# Autodesk Inventor assembly: Dropdown_Assembly_V3_Complete
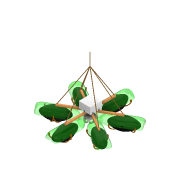
[picture p0: Inventor's stored thumbnail of the model, 180x180]
Saved by Autodesk Inventor 2021 (Build 250183000, 183)
## iProperties
Created: 2020-07-21
Part Number: Dropdown_Assembly_V3_Complete
Document SubType Name: Assembly
Designer: cameron
Mass: 991.522 g
Surface Area: 13651.5 cm^2
Volume: 1179.19 cm^3
Density: 0.840851 g/cm^3
Author: cameron
## Documents named in this file (10)
- C:\Users\camer\Git\Sure2020-DropdownSystem\InventorDropsonde\Dropdown_Assembly_V3_Complete.iam
- C:\Users\camer\Git\Sure2020-DropdownSystem\InventorDropsonde\PVC center piece.ipt
- C:\Users\camer\Git\Sure2020-DropdownSystem\InventorDropsonde\Dropdown_Assembly_V3.iam
- C:\Users\camer\Git\Sure2020-DropdownSystem\InventorDropsonde\Top rods.ipt
- C:\Users\camer\Git\Sure2020-DropdownSystem\InventorDropsonde\PCB housing.ipt
- C:\Users\camer\Git\Sure2020-DropdownSystem\InventorDropsonde\C brace.ipt
- C:\Users\camer\Git\Sure2020-DropdownSystem\InventorDropsonde\Balloon_Rope.ipt
- C:\Users\camer\OneDrive\Documents\Inventor\Content Center Files\R2021\en-US\AS 1427(04)\AS 1427 - M2.5 x 5(5) I.ipt
- C:\Users\camer\Git\Sure2020-DropdownSystem\InventorDropsonde\Staples.ipt
- C:\Users\camer\Git\Sure2020-DropdownSystem\InventorDropsonde\PCB_model_V5.ipt
## Components (29 placed, 9 different names)
1. PVC center piece:1 — Mate:1, Mate:2
2. Top rods:1 — Tangent:1, Tangent:2, Mate:3, Mate:4, Mate:6, Mate:8, Mate:10, Mate:12, Mate:14, Flush:1, Flush:2, Flush:10
3. PCB housing:1 — Mate:3, Mate:5, Mate:7, Mate:9, Mate:11, Mate:13, Mate:15, Mate:22
4. C brace:1 — Mate:10, Mate:11, Mate:16, Flush:7
5. C brace:2 — Mate:12, Mate:13, Mate:17, Flush:6
6. C brace:3 — Mate:4, Mate:5, Mate:18, Flush:8
7. C brace:4 — Mate:6, Mate:7, Mate:19, Flush:9
8. C brace:5 — Mate:8, Mate:9, Mate:20, Flush:4
9. C brace:6 — Mate:14, Mate:15, Mate:21, Flush:5
10. Balloon_Rope:1 — Flush:2, Flush:3
11. AS 1427 H - Metric M2.5 x 5:1 — Mate:16, Flush:7
12. AS 1427 H - Metric M2.5 x 5:2 — Mate:17, Flush:6
13. AS 1427 H - Metric M2.5 x 5:3 — Mate:18, Flush:8
14. AS 1427 H - Metric M2.5 x 5:4 — Mate:19, Flush:9
15. AS 1427 H - Metric M2.5 x 5:5 — Mate:20, Flush:4
16. AS 1427 H - Metric M2.5 x 5:6 — Mate:21, Flush:5
17. PCB_model_V5:1 — Mate:22
18. Dropdown_Assembly_V3:1 [sub-assembly] — Mate:1, Mate:2
19. Dropdown_Assembly_V3:2 [sub-assembly] — Tangent:2
20. Dropdown_Assembly_V3:3 [sub-assembly]
21. Dropdown_Assembly_V3:4 [sub-assembly] — Tangent:1
22. Dropdown_Assembly_V3:5 [sub-assembly]
23. Dropdown_Assembly_V3:6 [sub-assembly]
24. Staples:1 — Flush:11, Flush:12
25. Staples:2
26. Staples:3
27. Staples:4
28. Staples:5
29. Staples:6
## Component patterns: (6 elements, first: Dropdown_Assembly_V3:1), (6 elements, first: Staples:1)
## Relationships (36: Mate 22, Flush 12, Tangent 2)
- Mate:1: PVC center piece:1 ↔ Dropdown_Assembly_V3:1
- Mate:2: PVC center piece:1 ↔ Dropdown_Assembly_V3:1
- Tangent:1: Top rods:1 ↔ Dropdown_Assembly_V3:4
- Tangent:2: Top rods:1 ↔ Dropdown_Assembly_V3:2
- Mate:3 (1 mm): Top rods:1 ↔ PCB housing:1
- Mate:4: Top rods:1 ↔ C brace:3
- Mate:5: PCB housing:1 ↔ C brace:3
- Mate:6: Top rods:1 ↔ C brace:4
- Mate:7: PCB housing:1 ↔ C brace:4
- Mate:8: Top rods:1 ↔ C brace:5
- Mate:9: PCB housing:1 ↔ C brace:5
- Mate:10: Top rods:1 ↔ C brace:1
- Mate:11: PCB housing:1 ↔ C brace:1
- Mate:12: Top rods:1 ↔ C brace:2
- Mate:13: PCB housing:1 ↔ C brace:2
- Mate:14: Top rods:1 ↔ C brace:6
- Mate:15: PCB housing:1 ↔ C brace:6
- Flush:1 (300 mm): Top rods:1
- Flush:2: Top rods:1 ↔ Balloon_Rope:1
- Flush:3: Balloon_Rope:1
- Mate:16: C brace:1 ↔ AS 1427 H - Metric M2.5 x 5:1
- Mate:17: C brace:2 ↔ AS 1427 H - Metric M2.5 x 5:2
- Mate:18: C brace:3 ↔ AS 1427 H - Metric M2.5 x 5:3
- Mate:19: C brace:4 ↔ AS 1427 H - Metric M2.5 x 5:4
- Mate:20: C brace:5 ↔ AS 1427 H - Metric M2.5 x 5:5
- Mate:21: C brace:6 ↔ AS 1427 H - Metric M2.5 x 5:6
- Flush:4 (-0.25 mm): C brace:5 ↔ AS 1427 H - Metric M2.5 x 5:5
- Flush:5 (-0.25 mm): C brace:6 ↔ AS 1427 H - Metric M2.5 x 5:6
- Flush:6 (-0.25 mm): C brace:2 ↔ AS 1427 H - Metric M2.5 x 5:2
- Flush:7 (-0.25 mm): C brace:1 ↔ AS 1427 H - Metric M2.5 x 5:1
- Flush:8 (-0.25 mm): C brace:3 ↔ AS 1427 H - Metric M2.5 x 5:3
- Flush:9 (-0.25 mm): C brace:4 ↔ AS 1427 H - Metric M2.5 x 5:4
- Flush:10 (2 mm): Top rods:1
- Flush:11: Staples:1
- Flush:12: Staples:1
- Mate:22: PCB housing:1 ↔ PCB_model_V5:1
